# Autodesk Inventor assembly: Ankle
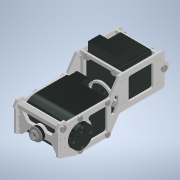
[picture p0: Inventor's stored thumbnail of the model, 180x180]
Saved by Autodesk Inventor 2020.4 (Build 244396000, 396)
## iProperties
Created: 2021-10-01
Part Number: Ankle
Document SubType Name: Assembly
Designer: Masato
Author: Masato
## Documents named in this file (15)
- C:\Users\Masato\Documents\Inventor\CIT Brains_Inventor\OpenPlatform_ver3_0（ワッシャ変更）\LowerBody\Ankle\Ankle.iam
- C:\Users\Masato\Documents\Inventor\CIT Brains_Inventor\OpenPlatform_ver3_0（ワッシャ変更）\Ready_Made\B3M10xx.ipt
- C:\Users\Masato\Documents\Inventor\CIT Brains_Inventor\OpenPlatform_ver3_0（ワッシャ変更）\Ready_Made\B3M11xx.ipt
- C:\Users\Masato\Documents\Inventor\CIT Brains_Inventor\OpenPlatform_ver3_0（ワッシャ変更）\Ready_Made\SLSBF6-39_5-M3-N3.ipt
- C:\Users\Masato\Documents\Inventor\CIT Brains_Inventor\OpenPlatform_ver3_0（ワッシャ変更）\Ready_Made\S3-07-3W.ipt
- C:\Users\Masato\Documents\Inventor\CIT Brains_Inventor\OpenPlatform_ver3_0（ワッシャ変更）\Ready_Made\UUW-0312-10BH.ipt
- C:\Users\Masato\Documents\Inventor\CIT Brains_Inventor\OpenPlatform_ver3_0（ワッシャ変更）\LowerBody\Ankle\Ankle_back_frame.ipt
- C:\Users\Masato\Documents\Inventor\CIT Brains_Inventor\OpenPlatform_ver3_0（ワッシャ変更）\LowerBody\Ankle\Ankle_front_frame.ipt
- C:\Users\Masato\Documents\Inventor\CIT Brains_Inventor\OpenPlatform_ver3_0（ワッシャ変更）\LowerBody\Ankle\Ankle_side_frame.ipt
- C:\Users\Masato\Documents\Inventor\CIT Brains_Inventor\OpenPlatform_ver3_0（ワッシャ変更）\Ready_Made\Screw\M2_6-15.ipt
- C:\Users\Masato\Documents\Inventor\CIT Brains_Inventor\OpenPlatform_ver3_0（ワッシャ変更）\Ready_Made\Screw\M2_6-20.ipt
- C:\Users\Masato\Documents\Inventor\CIT Brains_Inventor\OpenPlatform_ver3_0（ワッシャ変更）\Ready_Made\Screw\M3-6.ipt
- C:\Users\Masato\Documents\Inventor\CIT Brains_Inventor\OpenPlatform_ver3_0（ワッシャ変更）\Ready_Made\80F-0603.ipt
- C:\Users\Masato\Documents\Inventor\CIT Brains_Inventor\OpenPlatform_ver3_0（ワッシャ変更）\Ready_Made\free_horn.ipt
- C:\Users\Masato\Documents\Inventor\CIT Brains_Inventor\OpenPlatform_ver3_0（ワッシャ変更）\Ready_Made\CC-0612-15B.ipt
## Components (34 placed, 14 different names)
1. B3M10xx:1 — 挿入:15, 挿入:16, 挿入:17, 挿入:18, 挿入:43, 挿入:44, 挿入:45, 挿入:46
2. B3M11xx:1 — 挿入:1, 挿入:2, 挿入:3, 挿入:4, 挿入:5, 挿入:6, 挿入:7, 挿入:8, フラッシュ:4, メイト:3, フラッシュ:5, 挿入:42
3. SLSBF6-39_5-M3-N3:1 — 挿入:9, 挿入:10, 角度:2
4. SLSBF6-39_5-M3-N3:2 — 挿入:11, 挿入:12, 角度:3
5. S3-07-3W:1 — 角度:1, 挿入:19
6. UUW-0312-10BH:1 — 挿入:20, 挿入:51
7. Ankle_back_frame:1 — 挿入:15, 挿入:16, 挿入:17, 挿入:18, メイト:7, メイト:6, フラッシュ:3, 挿入:37, 挿入:38, 挿入:39, 挿入:40, 角度:3
8. Ankle_front_frame:1 — 角度:1, 挿入:19, 挿入:20, メイト:4, メイト:5, フラッシュ:1, 角度:2
9. Ankle_side_frame:1 — 挿入:5, 挿入:6, 挿入:7, 挿入:8, 挿入:10, 挿入:12, メイト:4, メイト:5, フラッシュ:1, 挿入:23, 挿入:24, 挿入:25, 挿入:26, 挿入:31, 挿入:32, メイト:7, メイト:6, フラッシュ:3
10. Ankle_side_frame:2 — 挿入:1, 挿入:2, 挿入:3, 挿入:4, 挿入:9, 挿入:11, 挿入:27, 挿入:28, 挿入:29, 挿入:30, 挿入:33, 挿入:34
11. M2_6-15:1 — 挿入:26
12. M2_6-15:2 — 挿入:25
13. M2_6-15:3 — 挿入:24
14. M2_6-15:4 — 挿入:23
15. M2_6-20:1 — 挿入:27
16. M2_6-20:2 — 挿入:28
17. M2_6-20:3 — 挿入:29
18. M2_6-20:4 — 挿入:30
19. M3-6:1 — 挿入:31
20. M3-6:2 — 挿入:32
21. M3-6:3 — 挿入:33
22. M3-6:4 — 挿入:34
23. M2_6-20:5 — 挿入:47
24. M2_6-20:6 — 挿入:50
25. M2_6-15:5 — 挿入:37
26. M2_6-15:6 — 挿入:38
27. M2_6-15:7 — 挿入:39
28. M2_6-15:8 — 挿入:40
29. 80F-0603:1 — 挿入:52
30. free_horn:1 — 挿入:42
31. Ankle_back_frame:2 — 挿入:43, 挿入:44, 挿入:45, 挿入:46, 挿入:47, 挿入:48, 挿入:49, 挿入:50
32. M2_6-20:7 — 挿入:48
33. M2_6-20:8 — 挿入:49
34. CC-0612-15B:1 — 挿入:51, 挿入:52
## Relationships (57: Insert 45, Mate 5, Flush 4, Angle 3)
- 挿入:1 [Insert]: B3M11xx:1 ↔ Ankle_side_frame:2
- 挿入:2 [Insert]: B3M11xx:1 ↔ Ankle_side_frame:2
- 挿入:3 [Insert]: B3M11xx:1 ↔ Ankle_side_frame:2
- 挿入:4 [Insert]: B3M11xx:1 ↔ Ankle_side_frame:2
- 挿入:5 [Insert]: B3M11xx:1 ↔ Ankle_side_frame:1
- 挿入:6 [Insert]: B3M11xx:1 ↔ Ankle_side_frame:1
- 挿入:7 [Insert]: B3M11xx:1 ↔ Ankle_side_frame:1
- 挿入:8 [Insert]: B3M11xx:1 ↔ Ankle_side_frame:1
- 挿入:9 [Insert]: SLSBF6-39_5-M3-N3:1 ↔ Ankle_side_frame:2
- 挿入:10 [Insert]: SLSBF6-39_5-M3-N3:1 ↔ Ankle_side_frame:1
- 挿入:11 [Insert]: SLSBF6-39_5-M3-N3:2 ↔ Ankle_side_frame:2
- 挿入:12 [Insert]: SLSBF6-39_5-M3-N3:2 ↔ Ankle_side_frame:1
- 挿入:15 [Insert]: B3M10xx:1 ↔ Ankle_back_frame:1
- 挿入:16 [Insert]: B3M10xx:1 ↔ Ankle_back_frame:1
- 挿入:17 [Insert]: B3M10xx:1 ↔ Ankle_back_frame:1
- 挿入:18 [Insert]: B3M10xx:1 ↔ Ankle_back_frame:1
- 角度:1 [Angle] (0 deg): S3-07-3W:1 ↔ Ankle_front_frame:1
- 挿入:19 [Insert]: S3-07-3W:1 ↔ Ankle_front_frame:1
- 挿入:20 [Insert]: UUW-0312-10BH:1 ↔ Ankle_front_frame:1
- フラッシュ:4 [Flush]: B3M11xx:1
- メイト:3 [Mate]: B3M11xx:1
- メイト:4 [Mate] (0.01 mm): Ankle_front_frame:1 ↔ Ankle_side_frame:1
- メイト:5 [Mate] (0.01 mm): Ankle_front_frame:1 ↔ Ankle_side_frame:1
- フラッシュ:1 [Flush]: Ankle_front_frame:1 ↔ Ankle_side_frame:1
- 角度:2 [Angle] (0 deg): SLSBF6-39_5-M3-N3:1 ↔ Ankle_front_frame:1
- 挿入:23 [Insert]: Ankle_side_frame:1 ↔ M2_6-15:4
- 挿入:24 [Insert]: Ankle_side_frame:1 ↔ M2_6-15:3
- 挿入:25 [Insert]: Ankle_side_frame:1 ↔ M2_6-15:2
- 挿入:26 [Insert]: Ankle_side_frame:1 ↔ M2_6-15:1
- 挿入:27 [Insert]: Ankle_side_frame:2 ↔ M2_6-20:1
- 挿入:28 [Insert]: Ankle_side_frame:2 ↔ M2_6-20:2
- 挿入:29 [Insert]: Ankle_side_frame:2 ↔ M2_6-20:3
- 挿入:30 [Insert]: Ankle_side_frame:2 ↔ M2_6-20:4
- 挿入:31 [Insert]: Ankle_side_frame:1 ↔ M3-6:1
- 挿入:32 [Insert]: Ankle_side_frame:1 ↔ M3-6:2
- 挿入:33 [Insert]: Ankle_side_frame:2 ↔ M3-6:3
- 挿入:34 [Insert]: Ankle_side_frame:2 ↔ M3-6:4
- メイト:7 [Mate] (0.01 mm): Ankle_back_frame:1 ↔ Ankle_side_frame:1
- メイト:6 [Mate] (0.01 mm): Ankle_back_frame:1 ↔ Ankle_side_frame:1
- フラッシュ:3 [Flush]: Ankle_back_frame:1 ↔ Ankle_side_frame:1
- 挿入:37 [Insert]: Ankle_back_frame:1 ↔ M2_6-15:5
- 挿入:38 [Insert]: Ankle_back_frame:1 ↔ M2_6-15:6
- 挿入:39 [Insert]: Ankle_back_frame:1 ↔ M2_6-15:7
- 挿入:40 [Insert]: Ankle_back_frame:1 ↔ M2_6-15:8
- 角度:3 [Angle] (0 deg): SLSBF6-39_5-M3-N3:2 ↔ Ankle_back_frame:1
- フラッシュ:5 [Flush] (-19.75 mm): B3M11xx:1
- 挿入:42 [Insert]: B3M11xx:1 ↔ free_horn:1
- 挿入:43 [Insert]: B3M10xx:1 ↔ Ankle_back_frame:2
- 挿入:44 [Insert]: B3M10xx:1 ↔ Ankle_back_frame:2
- 挿入:45 [Insert]: B3M10xx:1 ↔ Ankle_back_frame:2
- 挿入:46 [Insert]: B3M10xx:1 ↔ Ankle_back_frame:2
- 挿入:47 [Insert]: M2_6-20:5 ↔ Ankle_back_frame:2
- 挿入:48 [Insert]: Ankle_back_frame:2 ↔ M2_6-20:7
- 挿入:49 [Insert]: Ankle_back_frame:2 ↔ M2_6-20:8
- 挿入:50 [Insert]: M2_6-20:6 ↔ Ankle_back_frame:2
- 挿入:51 [Insert]: UUW-0312-10BH:1 ↔ CC-0612-15B:1
- 挿入:52 [Insert]: 80F-0603:1 ↔ CC-0612-15B:1
